# Autodesk Inventor assembly: ASY GNH 010 Dilution point
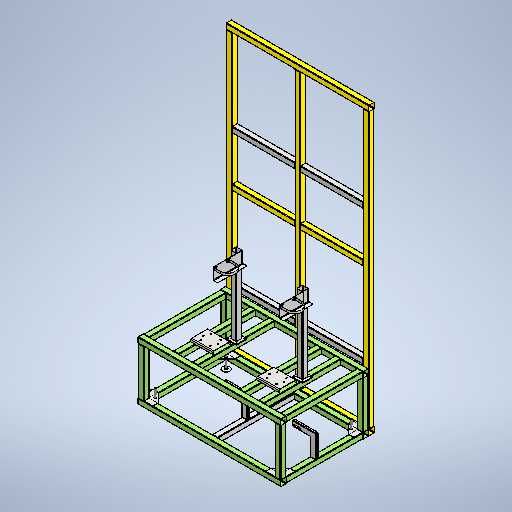
[picture p0: Inventor's stored thumbnail of the model, 512x512]
Saved by Autodesk Inventor 2025.1 (Build 291241020, 241B)
## iProperties
Created: 2025-03-06
Part Number: ASY GNH 010 Dilution point
Document SubType Name: Assembly
Designer: user
Mass: 85620.8 g
Surface Area: 87810.5 cm^2
Volume: 32343 cm^3
Density: 2.64727 g/cm^3
Author: user
## Documents named in this file (7)
- C:\Users\user\YandexDisk-badmisterfox\home pc\Inventor\GNH-Petrodvorec\ASY GNH 010 Dilution point.iam
- C:\Users\user\YandexDisk-badmisterfox\home pc\Inventor\GNH-Petrodvorec\ASY GNH 011 Dilution point Frame1.iam
- C:\Users\user\YandexDisk-badmisterfox\home pc\Inventor\GNH-Petrodvorec\ASY GNH 012 Dilution point Frame2.iam
- C:\Users\user\YandexDisk-badmisterfox\home pc\Inventor\GNH-Petrodvorec\TM06198C pump.ipt
- C:\Users\user\YandexDisk-badmisterfox\home pc\Inventor\GNH-Petrodvorec\Pulse compensator.ipt
- C:\Users\user\YandexDisk-badmisterfox\home pc\Inventor\GNH-Petrodvorec\BVI10(30)+EAQ-MINI220В-3Dвид-Вид1\BVI10(30)+EAQ-MINI220В-3Dвид-Вид1\BVI10(30)+EAQ-MINI220В-3Dвид-Вид1.ipt
- C:\Users\user\YandexDisk-badmisterfox\home pc\Inventor\GNH-Petrodvorec\Dummy chute.ipt
## Components (9 placed, 6 different names)
1. ASY GNH 011 Dilution point Frame1:1 [sub-assembly] — Rigid:2, Mate:1, Rigid:3
2. ASY GNH 012 Dilution point Frame2:1 [sub-assembly]
3. TM06198C pump:1 — Rigid:2, Cylindrical:1, Rigid:5
4. Pulse compensator:1 — Cylindrical:1, Mate:1, Flush:1
5. TM06198C pump:2 — Rigid:3, Rigid:4
6. Pulse compensator:2 — Flush:1
7. BVI10(30)+EAQ-MINI220В-3Dвид-Вид1:1 — Rigid:4
8. BVI10(30)+EAQ-MINI220В-3Dвид-Вид1:2 — Rigid:5
9. Dummy chute:1
## Relationships (9: WeldJoint 5, CylindricalJoint 2, Mate 1, Flush 1)
- [WeldJoint]: ASY GNH 011 Dilution point Frame1:1 ↔ ASY GNH 012 Dilution point Frame2:1
- Rigid:2 [WeldJoint]: ASY GNH 011 Dilution point Frame1:1 ↔ TM06198C pump:1
- Cylindrical:1: TM06198C pump:1 ↔ Pulse compensator:1
- Mate:1 (450 mm): ASY GNH 011 Dilution point Frame1:1 ↔ Pulse compensator:1
- [CylindricalJoint]: TM06198C pump:2 ↔ Pulse compensator:2
- Rigid:3 [WeldJoint]: ASY GNH 011 Dilution point Frame1:1 ↔ TM06198C pump:2
- Flush:1: Pulse compensator:1 ↔ Pulse compensator:2
- Rigid:4 [WeldJoint] (150 mm): TM06198C pump:2 ↔ BVI10(30)+EAQ-MINI220В-3Dвид-Вид1:1
- Rigid:5 [WeldJoint] (150 mm): TM06198C pump:1 ↔ BVI10(30)+EAQ-MINI220В-3Dвид-Вид1:2
## Named parameters: d5_d2 = -67.58804 deg, d6_d3 = 205 mm
